# Autodesk Inventor assembly: BoardAssembly
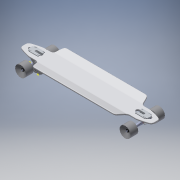
[picture p0: Inventor's stored thumbnail of the model, 180x180]
Saved by Autodesk Inventor 2018 (Build 220112000, 112)
## iProperties
Created: 2019-06-09
Part Number: BoardAssembly
Document SubType Name: Assembly
Designer: anirudh
Author: anirudh
## Documents named in this file (13)
- C:\Users\anirudh\Documents\MARS Fund\Electrical Skateboard\BoardAssembly.iam
- C:\Users\anirudh\Documents\MARS Fund\Electrical Skateboard\180mmParisTrucks\180mmParisTruck.iam
- C:\Users\anirudh\Documents\MARS Fund\Electrical Skateboard\WheelAssembly\WheelAssembly.iam
- C:\Users\anirudh\Documents\MARS Fund\Electrical Skateboard\MotorModel.ipt
- C:\Users\anirudh\Documents\MARS Fund\Electrical Skateboard\MotorBracket2.ipt
- C:\Users\anirudh\Documents\MARS Fund\Electrical Skateboard\Deck\DropThroughDeck.ipt
- C:\Users\anirudh\Documents\MARS Fund\Electrical Skateboard\MotorBracket3.ipt
- C:\Users\anirudh\Documents\MARS Fund\Electrical Skateboard\WheelGear.ipt
- C:\Users\anirudh\Documents\MARS Fund\Electrical Skateboard\MotorGear.ipt
- C:\Users\anirudh\Documents\MARS Fund\Electrical Skateboard\WheelAssembly\85mmWheel.ipt
- C:\Users\anirudh\Documents\MARS Fund\Electrical Skateboard\WheelAssembly\Skate-Bearing.ipt
- C:\Users\anirudh\Documents\MARS Fund\Electrical Skateboard\MotorGearCover.ipt
- C:\Users\anirudh\Documents\MARS Fund\Electrical Skateboard\MotorGearCover2.ipt
## Components (19 placed, 12 different names)
1. 180mmParisTruck:1 [sub-assembly] — Mate:21, Mate:22, Mate:23, Mate:33, Mate:34, Mate:36, Mate:37, Mate:40, Mate:41, Mate:44, Mate:46
2. 180mmParisTruck:2 [sub-assembly] — Mate:11, Mate:12, Mate:13, Mate:14, Mate:20, Mate:24, Mate:25
3. WheelAssembly:2 [sub-assembly] — Mate:13, Mate:14
4. WheelAssembly:3 [sub-assembly] — Mate:11, Mate:12
5. MotorModel:1 — Mate:15, Mate:16, Mate:30, Mate:43, Mate:51, Mate:53
6. MotorModel:2 — Mate:15, Mate:16, Mate:18, Mate:19, Mate:31, Mate:48, Mate:50
7. MotorBracket2:1 — Mate:18, Mate:19, Mate:26, Mate:27, Mate:28, Flush:1, Mate:39, Mate:49, Flush:2
8. DropThroughDeck:1 — Mate:20, Mate:21, Mate:22, Mate:23, Mate:24, Mate:25, Mate:26, Mate:27, Mate:28, Mate:29
9. MotorBracket3:1 — Mate:29, Mate:30, Flush:1, Mate:42, Mate:52, Flush:3
10. WheelGear:1 — Mate:33, Mate:34, Mate:35
11. MotorGear:1 — Mate:31, Mate:39
12. 85mmWheel:1 — Mate:35, Mate:36, Mate:38
13. Skate-Bearing:1 — Mate:37, Mate:38
14. MotorGear:2 — Mate:42, Mate:43
15. WheelGear:2 — Mate:40, Mate:41, Mate:45
16. 85mmWheel:2 — Mate:44, Mate:45, Mate:47
17. Skate-Bearing:2 — Mate:46, Mate:47
18. MotorGearCover:1 — Mate:48, Mate:49, Flush:2, Mate:50
19. MotorGearCover2:1 — Mate:51, Mate:52, Flush:3, Mate:53
## Relationships (44: Mate 41, Flush 3)
- Mate:11: 180mmParisTruck:2 ↔ WheelAssembly:3
- Mate:12: 180mmParisTruck:2 ↔ WheelAssembly:3
- Mate:13: 180mmParisTruck:2 ↔ WheelAssembly:2
- Mate:14: 180mmParisTruck:2 ↔ WheelAssembly:2
- Mate:15 (4.318 mm): MotorModel:1 ↔ MotorModel:2
- Mate:16: MotorModel:1 ↔ MotorModel:2
- Mate:18: MotorModel:2 ↔ MotorBracket2:1
- Mate:19: MotorModel:2 ↔ MotorBracket2:1
- Mate:20: 180mmParisTruck:2 ↔ DropThroughDeck:1
- Mate:21: 180mmParisTruck:1 ↔ DropThroughDeck:1
- Mate:22: 180mmParisTruck:1 ↔ DropThroughDeck:1
- Mate:23: 180mmParisTruck:1 ↔ DropThroughDeck:1
- Mate:24: 180mmParisTruck:2 ↔ DropThroughDeck:1
- Mate:25: 180mmParisTruck:2 ↔ DropThroughDeck:1
- Mate:26: MotorBracket2:1 ↔ DropThroughDeck:1
- Mate:27: MotorBracket2:1 ↔ DropThroughDeck:1
- Mate:28: MotorBracket2:1 ↔ DropThroughDeck:1
- Mate:29: DropThroughDeck:1 ↔ MotorBracket3:1
- Mate:30: MotorModel:1 ↔ MotorBracket3:1
- Flush:1: MotorBracket2:1 ↔ MotorBracket3:1
- Mate:31: MotorModel:2 ↔ MotorGear:1
- Mate:33: 180mmParisTruck:1 ↔ WheelGear:1
- Mate:34: 180mmParisTruck:1 ↔ WheelGear:1
- Mate:35: WheelGear:1 ↔ 85mmWheel:1
- Mate:36: 180mmParisTruck:1 ↔ 85mmWheel:1
- Mate:37: 180mmParisTruck:1 ↔ Skate-Bearing:1
- Mate:38: 85mmWheel:1 ↔ Skate-Bearing:1
- Mate:39 (0.5 mm): MotorBracket2:1 ↔ MotorGear:1
- Mate:40: 180mmParisTruck:1 ↔ WheelGear:2
- Mate:41: 180mmParisTruck:1 ↔ WheelGear:2
- Mate:42 (0.5 mm): MotorBracket3:1 ↔ MotorGear:2
- Mate:43: MotorModel:1 ↔ MotorGear:2
- Mate:44: 180mmParisTruck:1 ↔ 85mmWheel:2
- Mate:45: WheelGear:2 ↔ 85mmWheel:2
- Mate:46: 180mmParisTruck:1 ↔ Skate-Bearing:2
- Mate:47: 85mmWheel:2 ↔ Skate-Bearing:2
- Mate:48: MotorModel:2 ↔ MotorGearCover:1
- Mate:49: MotorBracket2:1 ↔ MotorGearCover:1
- Flush:2: MotorBracket2:1 ↔ MotorGearCover:1
- Mate:50: MotorModel:2 ↔ MotorGearCover:1
- Mate:51: MotorModel:1 ↔ MotorGearCover2:1
- Mate:52: MotorBracket3:1 ↔ MotorGearCover2:1
- Flush:3: MotorBracket3:1 ↔ MotorGearCover2:1
- Mate:53: MotorModel:1 ↔ MotorGearCover2:1
